# Autodesk Inventor assembly: Main Assembly
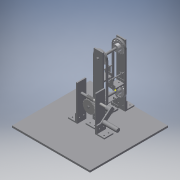
[picture p0: Inventor's stored thumbnail of the model, 180x180]
Saved by Autodesk Inventor 2018 (Build 220112000, 112)
## iProperties
Created: 2017-04-14
Part Number: Main Assembly
Document SubType Name: Assembly
Designer: Administrator
Author: Administrator
## Documents named in this file (13)
- C:\Users\Administrator\Documents\TA202\Main Assembly.iam
- C:\Users\Administrator\Documents\TA202\Angle.ipt
- C:\Users\Administrator\Documents\TA202\Main Support.ipt
- C:\Users\Administrator\Documents\TA202\Sprocket Axle.ipt
- C:\Users\Administrator\Documents\TA202\Sprocket.ipt
- C:\Users\Administrator\Documents\TA202\Worm Gear.ipt
- C:\Users\Administrator\Documents\TA202\Worm Axle.ipt
- C:\Users\Administrator\Documents\TA202\Worm.ipt
- C:\Users\Administrator\Documents\TA202\Worm Support.ipt
- C:\Users\Administrator\Documents\TA202\Base Plate.ipt
- C:\Users\Administrator\Documents\TA202\Bed Plate Assembly.iam
- C:\Users\Administrator\Documents\TA202\Chain.ipt
- C:\Users\Administrator\Documents\TA202\Handle Assembly.iam
## Components (23 placed, 12 different names)
1. Angle:1 — Mate:1, Flush:1, Flush:3, Angle:1, Mate:4, Angle:4, Mate:18, Mate:21
2. Main Support:1 — Mate:1, Flush:1, Flush:3, Insert:2, Angle:3, Insert:10, Mate:19, Angle:15
3. Angle:2 — Flush:4, Angle:1, Flush:7, Mate:8, Mate:17, Mate:20, Mate:22
4. Main Support:2 — Flush:4, Insert:1, Insert:5, Mate:23
5. Sprocket Axle:1 — Insert:1, Insert:2, Insert:3, Insert:4, Insert:12, Insert:13, Angle:10, Angle:11
6. Sprocket:1 — Insert:3
7. Sprocket:2 — Insert:4
8. Worm Gear:1 — Insert:6
9. Worm Axle:1 — Insert:5, Insert:6, Insert:9
10. Worm:1 — Angle:3, Insert:7, Insert:8, Insert:17
11. Worm Support:1 — Mate:3, Flush:5, Flush:6, Insert:7, Mate:12
12. Angle:3 — Mate:3, Flush:5, Flush:6, Angle:4, Angle:5, Angle:6, Mate:7, Mate:9, Mate:10, Mate:11
13. Base Plate:1 — Mate:4, Flush:7, Angle:6, Mate:7, Mate:8, Angle:7, Angle:8, Angle:14, Mate:9, Mate:10, Mate:11, Mate:12, Mate:13, Mate:14, Mate:15, Mate:16, Mate:17, Mate:18, Mate:19, Mate:20, Mate:21, Mate:22, Mate:23, Angle:16
14. Worm Support:2 — Insert:8, Mate:16
15. Angle:4 — Angle:5, Mate:13, Mate:14, Mate:15
16. Sprocket:3 — Insert:9
17. Sprocket:4 — Insert:10
18. Bed Plate Assembly:1 [sub-assembly] — Angle:7, Angle:10, Insert:14
19. Bed Plate Assembly:3 [sub-assembly] — Angle:8, Angle:11, Insert:15
20. Chain:2 — Insert:12, Angle:13, Insert:14, Insert:15, Insert:16
21. Chain:3 — Insert:13, Angle:13, Angle:15
22. Bed Plate Assembly:4 [sub-assembly] — Insert:16, Angle:14
23. Handle Assembly:1 [sub-assembly] — Insert:17
## Relationships (60: Mate 22, Insert 16, Angle 13, Flush 9)
- Mate:1: Angle:1 ↔ Main Support:1
- Flush:1: Angle:1 ↔ Main Support:1
- [Mate]: Angle:2 ↔ Main Support:2
- [Flush]: Angle:2 ↔ Main Support:2
- Flush:3: Angle:1 ↔ Main Support:1
- Flush:4: Angle:2 ↔ Main Support:2
- Insert:1 (-15 mm): Main Support:2 ↔ Sprocket Axle:1
- Insert:2 (-15 mm): Main Support:1 ↔ Sprocket Axle:1
- Insert:3 (-43 mm): Sprocket Axle:1 ↔ Sprocket:1
- Insert:4 (-43 mm): Sprocket Axle:1 ↔ Sprocket:2
- Insert:5 (-15 mm): Main Support:2 ↔ Worm Axle:1
- Insert:6 (-20 mm): Worm Gear:1 ↔ Worm Axle:1
- Angle:1 (0 deg): Angle:1 ↔ Angle:2
- Angle:3 (90 deg): Main Support:1 ↔ Worm:1
- Mate:3: Worm Support:1 ↔ Angle:3
- Flush:5: Worm Support:1 ↔ Angle:3
- Flush:6: Worm Support:1 ↔ Angle:3
- Mate:4: Angle:1 ↔ Base Plate:1
- Flush:7: Angle:2 ↔ Base Plate:1
- Angle:4 (0 deg): Angle:1 ↔ Angle:3
- Insert:7 (-125 mm): Worm:1 ↔ Worm Support:1
- [Mate]: Worm Support:2 ↔ Angle:4
- [Flush]: Worm Support:2 ↔ Angle:4
- [Flush]: Worm Support:2 ↔ Angle:4
- Insert:8 (-19 mm): Worm:1 ↔ Worm Support:2
- Insert:9 (-43 mm): Worm Axle:1 ↔ Sprocket:3
- Insert:10 (-34 mm): Main Support:1 ↔ Sprocket:4
- Angle:5 (0 deg): Angle:3 ↔ Angle:4
- Angle:6 (0 deg): Angle:3 ↔ Base Plate:1
- Mate:7: Angle:3 ↔ Base Plate:1
- Mate:8: Angle:2 ↔ Base Plate:1
- Insert:12 (-132 mm): Sprocket Axle:1 ↔ Chain:2
- Insert:13 (-27 mm): Sprocket Axle:1 ↔ Chain:3
- Angle:7 (0 deg): Base Plate:1 ↔ Bed Plate Assembly:1
- Angle:8 (0 deg): Base Plate:1 ↔ Bed Plate Assembly:3
- Angle:10 (0 deg): Sprocket Axle:1 ↔ Bed Plate Assembly:1
- Angle:11 (0 deg): Sprocket Axle:1 ↔ Bed Plate Assembly:3
- Angle:13 (0 deg): Chain:2 ↔ Chain:3
- Insert:14 (5 mm): Bed Plate Assembly:1 ↔ Chain:2
- Insert:15 (5 mm): Bed Plate Assembly:3 ↔ Chain:2
- Insert:16 (5 mm): Chain:2 ↔ Bed Plate Assembly:4
- Angle:14 (0 deg): Base Plate:1 ↔ Bed Plate Assembly:4
- Mate:9: Angle:3 ↔ Base Plate:1
- Mate:10: Angle:3 ↔ Base Plate:1
- Mate:11: Angle:3 ↔ Base Plate:1
- Mate:12: Worm Support:1 ↔ Base Plate:1
- Mate:13: Base Plate:1 ↔ Angle:4
- Mate:14: Base Plate:1 ↔ Angle:4
- Mate:15: Base Plate:1 ↔ Angle:4
- Mate:16: Base Plate:1 ↔ Worm Support:2
- Mate:17: Angle:2 ↔ Base Plate:1
- Mate:18: Angle:1 ↔ Base Plate:1
- Mate:19: Main Support:1 ↔ Base Plate:1
- Mate:20: Angle:2 ↔ Base Plate:1
- Mate:21: Angle:1 ↔ Base Plate:1
- Mate:22: Angle:2 ↔ Base Plate:1
- Mate:23: Main Support:2 ↔ Base Plate:1
- Angle:15 (0 deg): Main Support:1 ↔ Chain:3
- Insert:17: Worm:1 ↔ Handle Assembly:1
- Angle:16 (0 deg): Base Plate:1
## Named parameters: d2_d0 = 0 mm, d3_d1 = 0 mm, d23_d15 = 0 mm, d24_d16 = 0 mm, d25_d17 = 0 mm
